# Autodesk Inventor assembly: ASY PNS680-Filter legs D1000
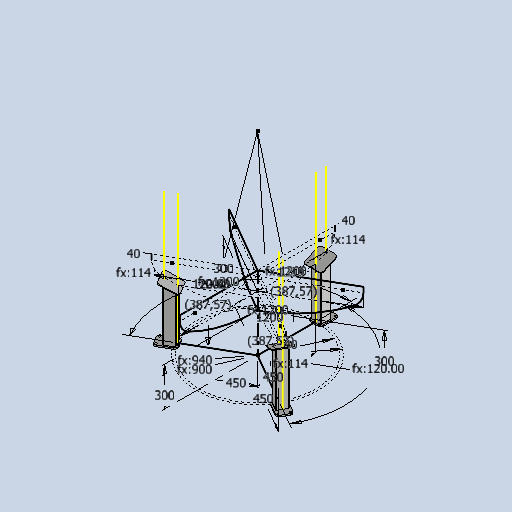
[picture p0: Inventor's stored thumbnail of the model, 512x512]
Saved by Autodesk Inventor 2025.1 (Build 291241020, 241B)
## iProperties
Created: 2025-02-20
Part Number: ASY PNS680-Filter legs D1000
Document SubType Name: Assembly
Designer: user
Author: user
## Documents named in this file (5)
- C:\Users\user\YandexDisk-badmisterfox\home pc\Inventor\Pressure-filters\D1200\ASY PNS680-Filter legs D1200.iam
- C:\Users\user\YandexDisk-badmisterfox\home pc\Inventor\Pressure-filters\Filter D1000\PNS-681 Leg tube.ipt
- C:\Users\user\YandexDisk-badmisterfox\home pc\Inventor\Pressure-filters\D1200\PNS-689 leg sketch.ipt
- C:\Users\user\YandexDisk-badmisterfox\home pc\Inventor\Pressure-filters\D1200\PNS-682 leg plate for filter.ipt
- C:\Users\user\YandexDisk-badmisterfox\home pc\Inventor\Pressure-filters\D1200\PNS-683 leg floor plate.ipt
## Components (10 placed, 4 different names)
1. PNS-681 Leg tube.ipt:1 — Mate:2, Mate:8, Tangent:2, Rigid:2, Rigid:5
2. PNS-681 Leg tube.ipt:2 — Mate:4, Mate:7, Tangent:3, Rigid:1, Rigid:4
3. PNS-681 Leg tube.ipt:3 — Mate:3, Mate:6, Tangent:1, Rigid:3, Rigid:6
4. PNS-689 leg sketch.ipt:1 — Mate:6, Tangent:1, Mate:7, Mate:8, Tangent:2, Tangent:3
5. PNS-682 leg plate for filter.ipt:1 — Rigid:1
6. PNS-682 leg plate for filter.ipt:2 — Rigid:2
7. PNS-682 leg plate for filter.ipt:3 — Rigid:3
8. PNS-683 leg floor plate.ipt:1 — Rigid:4
9. PNS-683 leg floor plate.ipt:2 — Rigid:5
10. PNS-683 leg floor plate.ipt:3 — Rigid:6
## Relationships (15: Mate 6, WeldJoint 6, Tangent 3)
- Mate:2: PNS-681 Leg tube.ipt:1
- Mate:3: PNS-681 Leg tube.ipt:3
- Mate:4: PNS-681 Leg tube.ipt:2
- Mate:6: PNS-681 Leg tube.ipt:3 ↔ PNS-689 leg sketch.ipt:1
- Tangent:1: PNS-681 Leg tube.ipt:3 ↔ PNS-689 leg sketch.ipt:1
- Mate:7: PNS-681 Leg tube.ipt:2 ↔ PNS-689 leg sketch.ipt:1
- Mate:8: PNS-681 Leg tube.ipt:1 ↔ PNS-689 leg sketch.ipt:1
- Tangent:2: PNS-681 Leg tube.ipt:1 ↔ PNS-689 leg sketch.ipt:1
- Tangent:3: PNS-681 Leg tube.ipt:2 ↔ PNS-689 leg sketch.ipt:1
- Rigid:1 [WeldJoint]: PNS-681 Leg tube.ipt:2 ↔ PNS-682 leg plate for filter.ipt:1
- Rigid:2 [WeldJoint]: PNS-681 Leg tube.ipt:1 ↔ PNS-682 leg plate for filter.ipt:2
- Rigid:3 [WeldJoint]: PNS-681 Leg tube.ipt:3 ↔ PNS-682 leg plate for filter.ipt:3
- Rigid:4 [WeldJoint]: PNS-681 Leg tube.ipt:2 ↔ PNS-683 leg floor plate.ipt:1
- Rigid:5 [WeldJoint]: PNS-681 Leg tube.ipt:1 ↔ PNS-683 leg floor plate.ipt:2
- Rigid:6 [WeldJoint]: PNS-681 Leg tube.ipt:3 ↔ PNS-683 leg floor plate.ipt:3
